# Autodesk Inventor assembly: Assembly1
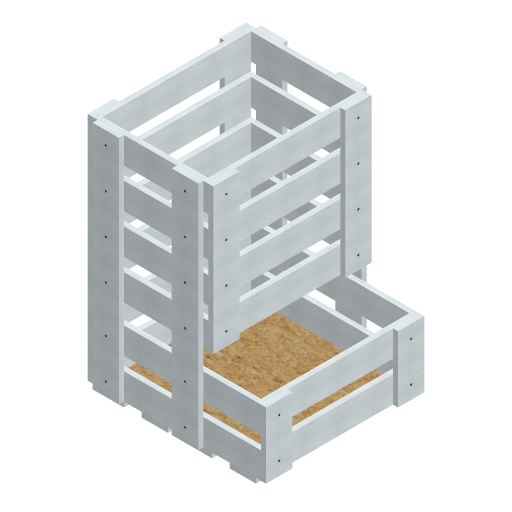
[picture p0: Inventor's stored thumbnail of the model, 512x512]
Saved by Autodesk Inventor 2024 (Build 280153000, 153)
## iProperties
Created: 2024-03-20
Part Number: Assembly1
Document SubType Name: Assembly
Designer: marco
Author: marco
## Documents named in this file (13)
- C:\Users\marco\OneDrive\Documents\FruitRack\Assembly1.iam
- C:\Users\marco\OneDrive\Documents\FruitRack\A.ipt
- C:\Users\marco\OneDrive\Documents\FruitRack\B.ipt
- C:\Users\marco\OneDrive\Documents\FruitRack\C.ipt
- C:\Users\marco\OneDrive\Documents\FruitRack\D.ipt
- C:\Users\marco\OneDrive\Documents\FruitRack\E.ipt
- C:\Users\marco\OneDrive\Documents\FruitRack\Screw.ipt
- C:\Users\marco\OneDrive\Documents\FruitRack\F.ipt
- C:\Users\marco\OneDrive\Documents\FruitRack\G.ipt
- C:\Users\marco\OneDrive\Documents\FruitRack\H.ipt
- C:\Users\marco\OneDrive\Documents\FruitRack\I.ipt
- C:\Users\marco\OneDrive\Documents\FruitRack\J.ipt
- C:\Users\marco\OneDrive\Documents\FruitRack\K.ipt
## Components (119 placed, 12 different names)
1. A:1 — Rigid:1, Rigid:2, Rigid:49, Rigid:68
2. A:2 — Rigid:3, Rigid:4, Rigid:50, Rigid:69
3. A:3 — Rigid:5, Rigid:6, Rigid:51, Rigid:70
4. A:4 — Rigid:7, Rigid:8, Rigid:52, Rigid:71
5. A:5 — Rigid:13, Rigid:14, Rigid:55, Rigid:62
6. A:6 — Rigid:15, Rigid:16, Rigid:56, Rigid:63
7. A:7 — Rigid:17, Rigid:18, Rigid:57, Rigid:64
8. A:8 — Rigid:19, Rigid:20, Rigid:58, Rigid:65
9. B:1 — Rigid:21, Rigid:22, Rigid:59, Rigid:66
10. B:2 — Rigid:9, Rigid:10, Rigid:53, Rigid:72
11. C:1 — Rigid:11, Rigid:12, Rigid:54, Rigid:73, Rigid:129, Rigid:130, Rigid:131, Rigid:132, Rigid:133
12. D:1 — Rigid:23, Rigid:24, Rigid:60, Rigid:67, Rigid:134, Rigid:135, Rigid:136, Rigid:137
13. E:1 — Rigid:25, Rigid:26, Rigid:27, Rigid:28, Rigid:29, Rigid:30
14. E:2 — Rigid:31, Rigid:32, Rigid:33, Rigid:34, Rigid:35, Rigid:36
15. E:3 — Rigid:43, Rigid:44, Rigid:45, Rigid:46, Rigid:47, Rigid:48
16. E:4 — Rigid:37, Rigid:38, Rigid:39, Rigid:40, Rigid:41, Rigid:42
17. Screw:1 — Rigid:1, Rigid:25
18. Screw:2 — Rigid:2, Rigid:31
19. Screw:3 — Rigid:3, Rigid:26
20. Screw:4 — Rigid:4, Rigid:32
21. Screw:5 — Rigid:5, Rigid:27
22. Screw:6 — Rigid:6, Rigid:33
23. Screw:7 — Rigid:7, Rigid:28
24. Screw:8 — Rigid:8, Rigid:34
25. Screw:9 — Rigid:9, Rigid:29
26. Screw:10 — Rigid:10, Rigid:35
27. Screw:11 — Rigid:11, Rigid:30
28. Screw:12 — Rigid:12, Rigid:36
29. Screw:13 — Rigid:13, Rigid:43
30. Screw:14 — Rigid:14, Rigid:37
31. Screw:15 — Rigid:15, Rigid:44
32. Screw:16 — Rigid:16, Rigid:38
33. Screw:17 — Rigid:17, Rigid:45
34. Screw:18 — Rigid:18, Rigid:39
35. Screw:19 — Rigid:19, Rigid:46
36. Screw:20 — Rigid:20, Rigid:40
37. Screw:21 — Rigid:21, Rigid:47
38. Screw:22 — Rigid:22, Rigid:41
39. Screw:23 — Rigid:23, Rigid:48
40. Screw:24 — Rigid:24, Rigid:42
41. F:1 — Rigid:74, Rigid:78, Rigid:87, Rigid:100
42. F:2 — Rotational:1, Rigid:79, Rigid:88, Rigid:94
43. F:3 — Rotational:2, Rigid:80, Rigid:89, Rigid:95
44. F:4 — Rigid:75, Rigid:90, Rigid:96
45. F:5 — Rigid:76, Rigid:91, Rigid:97
46. F:6 — Rigid:77, Rigid:98, Rigid:92
47. F:7 — Rotational:4, Rigid:110, Rigid:116
48. F:8 — Rigid:104, Rigid:111, Rigid:117
49. F:9 — Rigid:109, Rigid:112, Rigid:118
50. F:10 — Rigid:106, Rigid:113, Rigid:122
51. F:11 — Rigid:107, Rigid:114, Rigid:120
52. F:12 — Rigid:108, Rigid:115, Rigid:121
53. G:1 — Rigid:101
54. G:2 — Rigid:102
55. H:1 — Rotational:3
56. H:2 — Rigid:103
57. I:1 — Rigid:124, Rigid:125, Rigid:126, Rigid:127, Rigid:128
58. I:2 — Rigid:123
59. Screw:25 — Rigid:49, Rigid:74
60. Screw:26 — Rigid:50, Rotational:1
61. Screw:27 — Rigid:51, Rotational:2
62. Screw:28 — Rigid:52, Rigid:75
63. Screw:29 — Rigid:53, Rigid:76
64. Screw:30 — Rigid:54, Rigid:77
65. Screw:31 — Rigid:55, Rigid:78
66. Screw:32 — Rigid:56, Rigid:79
67. Screw:33 — Rigid:57, Rigid:80
68. Screw:34 — Rigid:58
69. Screw:35 — Rigid:59
70. Screw:36 — Rigid:60
71. Screw:37 — Rigid:68, Rotational:4
72. Screw:38 — Rigid:69, Rigid:104
73. Screw:39 — Rigid:70, Rigid:109
74. Screw:40 — Rigid:71, Rigid:106
75. Screw:41 — Rigid:72, Rigid:107
76. Screw:42 — Rigid:73, Rigid:108
77. Screw:43 — Rigid:63
78. Screw:44 — Rigid:62
79. Screw:45 — Rigid:64
80. Screw:46 — Rigid:65
81. Screw:47 — Rigid:66
82. Screw:48 — Rigid:67
83. Screw:49 — Rigid:87, Rigid:101
84. Screw:50 — Rigid:88
85. Screw:51 — Rigid:89
86. Screw:52 — Rigid:90
87. Screw:53 — Rigid:91, Rotational:3
88. Screw:54 — Rigid:92
89. Screw:55 — Rigid:100, Rigid:102
90. Screw:56 — Rigid:94
91. Screw:57 — Rigid:95
92. Screw:58 — Rigid:96
93. Screw:59 — Rigid:97, Rigid:103
94. Screw:60 — Rigid:98
95. Screw:61 — Rigid:110, Rigid:123
96. Screw:62 — Rigid:111
97. Screw:63 — Rigid:112
98. Screw:64 — Rigid:113
99. Screw:65 — Rigid:114
100. Screw:66 — Rigid:115
101. Screw:67 — Rigid:118, Rigid:127
102. Screw:68 — Rigid:116, Rigid:125
103. Screw:69 — Rigid:117, Rigid:126
104. Screw:70 — Rigid:122
105. Screw:71 — Rigid:120, Rigid:128
106. Screw:72 — Rigid:121, Rigid:124
107. J:1 — Rigid:138
108. J:2 — Rigid:139
109. J:3 — Rigid:140
110. J:4 — Rigid:141
111. K:1 — Rigid:129
112. Screw:73 — Rigid:130, Rigid:138
113. Screw:74 — Rigid:134
114. Screw:75 — Rigid:131, Rigid:139
115. Screw:76 — Rigid:135
116. Screw:77 — Rigid:132, Rigid:140
117. Screw:78 — Rigid:136
118. Screw:79 — Rigid:133, Rigid:141
119. Screw:80 — Rigid:137
## Relationships (134: WeldJoint 130, RevoluteJoint 4)
- Rigid:1 [WeldJoint] (11 mm): A:1 ↔ Screw:1
- Rigid:2 [WeldJoint] (11 mm): A:1 ↔ Screw:2
- Rigid:3 [WeldJoint] (11 mm): A:2 ↔ Screw:3
- Rigid:4 [WeldJoint] (11 mm): A:2 ↔ Screw:4
- Rigid:5 [WeldJoint] (11 mm): A:3 ↔ Screw:5
- Rigid:6 [WeldJoint] (11 mm): A:3 ↔ Screw:6
- Rigid:7 [WeldJoint] (11 mm): A:4 ↔ Screw:7
- Rigid:8 [WeldJoint] (11 mm): A:4 ↔ Screw:8
- Rigid:9 [WeldJoint] (11 mm): B:2 ↔ Screw:9
- Rigid:10 [WeldJoint] (11 mm): B:2 ↔ Screw:10
- Rigid:11 [WeldJoint] (11 mm): C:1 ↔ Screw:11
- Rigid:12 [WeldJoint] (11 mm): C:1 ↔ Screw:12
- Rigid:13 [WeldJoint] (11 mm): A:5 ↔ Screw:13
- Rigid:14 [WeldJoint] (11 mm): A:5 ↔ Screw:14
- Rigid:15 [WeldJoint] (11 mm): A:6 ↔ Screw:15
- Rigid:16 [WeldJoint] (11 mm): A:6 ↔ Screw:16
- Rigid:17 [WeldJoint] (11 mm): A:7 ↔ Screw:17
- Rigid:18 [WeldJoint] (11 mm): A:7 ↔ Screw:18
- Rigid:19 [WeldJoint] (11 mm): A:8 ↔ Screw:19
- Rigid:20 [WeldJoint] (11 mm): A:8 ↔ Screw:20
- Rigid:21 [WeldJoint] (11 mm): B:1 ↔ Screw:21
- Rigid:22 [WeldJoint] (11 mm): B:1 ↔ Screw:22
- Rigid:23 [WeldJoint] (11 mm): D:1 ↔ Screw:23
- Rigid:24 [WeldJoint] (11 mm): D:1 ↔ Screw:24
- Rigid:25 [WeldJoint]: E:1 ↔ Screw:1
- Rigid:26 [WeldJoint]: E:1 ↔ Screw:3
- Rigid:27 [WeldJoint]: E:1 ↔ Screw:5
- Rigid:28 [WeldJoint]: E:1 ↔ Screw:7
- Rigid:29 [WeldJoint]: E:1 ↔ Screw:9
- Rigid:30 [WeldJoint]: E:1 ↔ Screw:11
- Rigid:31 [WeldJoint]: E:2 ↔ Screw:2
- Rigid:32 [WeldJoint]: E:2 ↔ Screw:4
- Rigid:33 [WeldJoint]: E:2 ↔ Screw:6
- Rigid:34 [WeldJoint]: E:2 ↔ Screw:8
- Rigid:35 [WeldJoint]: E:2 ↔ Screw:10
- Rigid:36 [WeldJoint]: E:2 ↔ Screw:12
- Rigid:37 [WeldJoint]: E:4 ↔ Screw:14
- Rigid:38 [WeldJoint]: E:4 ↔ Screw:16
- Rigid:39 [WeldJoint]: E:4 ↔ Screw:18
- Rigid:40 [WeldJoint]: E:4 ↔ Screw:20
- Rigid:41 [WeldJoint]: E:4 ↔ Screw:22
- Rigid:42 [WeldJoint]: E:4 ↔ Screw:24
- Rigid:43 [WeldJoint]: E:3 ↔ Screw:13
- Rigid:44 [WeldJoint]: E:3 ↔ Screw:15
- Rigid:45 [WeldJoint]: E:3 ↔ Screw:17
- Rigid:46 [WeldJoint]: E:3 ↔ Screw:19
- Rigid:47 [WeldJoint]: E:3 ↔ Screw:21
- Rigid:48 [WeldJoint]: E:3 ↔ Screw:23
- Rigid:49 [WeldJoint]: A:1 ↔ Screw:25
- Rigid:50 [WeldJoint]: A:2 ↔ Screw:26
- Rigid:51 [WeldJoint]: A:3 ↔ Screw:27
- Rigid:52 [WeldJoint]: A:4 ↔ Screw:28
- Rigid:53 [WeldJoint]: B:2 ↔ Screw:29
- Rigid:54 [WeldJoint]: C:1 ↔ Screw:30
- Rigid:55 [WeldJoint]: A:5 ↔ Screw:31
- Rigid:56 [WeldJoint]: A:6 ↔ Screw:32
- Rigid:58 [WeldJoint]: A:8 ↔ Screw:34
- Rigid:59 [WeldJoint]: B:1 ↔ Screw:35
- Rigid:60 [WeldJoint]: D:1 ↔ Screw:36
- Rigid:57 [WeldJoint]: A:7 ↔ Screw:33
- Rigid:62 [WeldJoint]: A:5 ↔ Screw:44
- Rigid:63 [WeldJoint]: A:6 ↔ Screw:43
- Rigid:64 [WeldJoint]: A:7 ↔ Screw:45
- Rigid:65 [WeldJoint]: A:8 ↔ Screw:46
- Rigid:66 [WeldJoint]: B:1 ↔ Screw:47
- Rigid:67 [WeldJoint]: D:1 ↔ Screw:48
- Rigid:68 [WeldJoint]: A:1 ↔ Screw:37
- Rigid:69 [WeldJoint]: A:2 ↔ Screw:38
- Rigid:70 [WeldJoint]: A:3 ↔ Screw:39
- Rigid:71 [WeldJoint]: A:4 ↔ Screw:40
- Rigid:72 [WeldJoint]: B:2 ↔ Screw:41
- Rigid:73 [WeldJoint]: C:1 ↔ Screw:42
- Rigid:74 [WeldJoint]: F:1 ↔ Screw:25
- Rotational:1 [RevoluteJoint]: F:2 ↔ Screw:26
- Rotational:2 [RevoluteJoint]: F:3 ↔ Screw:27
- Rigid:75 [WeldJoint]: F:4 ↔ Screw:28
- Rigid:76 [WeldJoint]: F:5 ↔ Screw:29
- Rigid:77 [WeldJoint]: F:6 ↔ Screw:30
- Rigid:78 [WeldJoint]: F:1 ↔ Screw:31
- Rigid:79 [WeldJoint]: F:2 ↔ Screw:32
- Rigid:80 [WeldJoint]: F:3 ↔ Screw:33
- Rigid:87 [WeldJoint]: F:1 ↔ Screw:49
- Rigid:88 [WeldJoint]: F:2 ↔ Screw:50
- Rigid:89 [WeldJoint]: F:3 ↔ Screw:51
- Rigid:90 [WeldJoint]: F:4 ↔ Screw:52
- Rigid:91 [WeldJoint]: F:5 ↔ Screw:53
- Rigid:94 [WeldJoint]: F:2 ↔ Screw:56
- Rigid:95 [WeldJoint]: F:3 ↔ Screw:57
- Rigid:96 [WeldJoint]: F:4 ↔ Screw:58
- Rigid:97 [WeldJoint]: F:5 ↔ Screw:59
- Rigid:98 [WeldJoint]: F:6 ↔ Screw:60
- Rigid:92 [WeldJoint]: F:6 ↔ Screw:54
- Rigid:100 [WeldJoint]: F:1 ↔ Screw:55
- Rigid:101 [WeldJoint]: G:1 ↔ Screw:49
- Rigid:102 [WeldJoint]: G:2 ↔ Screw:55
- Rigid:103 [WeldJoint]: H:2 ↔ Screw:59
- Rotational:3 [RevoluteJoint]: H:1 ↔ Screw:53
- Rotational:4 [RevoluteJoint]: F:7 ↔ Screw:37
- Rigid:104 [WeldJoint]: F:8 ↔ Screw:38
- Rigid:106 [WeldJoint]: F:10 ↔ Screw:40
- Rigid:107 [WeldJoint]: F:11 ↔ Screw:41
- Rigid:108 [WeldJoint]: F:12 ↔ Screw:42
- Rigid:109 [WeldJoint]: F:9 ↔ Screw:39
- Rigid:110 [WeldJoint]: F:7 ↔ Screw:61
- Rigid:111 [WeldJoint]: F:8 ↔ Screw:62
- Rigid:112 [WeldJoint]: F:9 ↔ Screw:63
- Rigid:113 [WeldJoint]: F:10 ↔ Screw:64
- Rigid:114 [WeldJoint]: F:11 ↔ Screw:65
- Rigid:115 [WeldJoint]: F:12 ↔ Screw:66
- Rigid:116 [WeldJoint]: F:7 ↔ Screw:68
- Rigid:117 [WeldJoint]: F:8 ↔ Screw:69
- Rigid:118 [WeldJoint]: F:9 ↔ Screw:67
- Rigid:120 [WeldJoint]: F:11 ↔ Screw:71
- Rigid:121 [WeldJoint]: F:12 ↔ Screw:72
- Rigid:122 [WeldJoint]: F:10 ↔ Screw:70
- Rigid:123 [WeldJoint]: I:2 ↔ Screw:61
- Rigid:124 [WeldJoint]: I:1 ↔ Screw:72
- Rigid:125 [WeldJoint]: I:1 ↔ Screw:68
- Rigid:126 [WeldJoint]: I:1 ↔ Screw:69
- Rigid:127 [WeldJoint]: I:1 ↔ Screw:67
- Rigid:128 [WeldJoint]: I:1 ↔ Screw:71
- Rigid:129 [WeldJoint]: C:1 ↔ K:1
- Rigid:130 [WeldJoint]: C:1 ↔ Screw:73
- Rigid:131 [WeldJoint]: C:1 ↔ Screw:75
- Rigid:132 [WeldJoint]: C:1 ↔ Screw:77
- Rigid:133 [WeldJoint]: C:1 ↔ Screw:79
- Rigid:134 [WeldJoint]: D:1 ↔ Screw:74
- Rigid:135 [WeldJoint]: D:1 ↔ Screw:76
- Rigid:136 [WeldJoint]: D:1 ↔ Screw:78
- Rigid:137 [WeldJoint]: D:1 ↔ Screw:80
- Rigid:138 [WeldJoint]: J:1 ↔ Screw:73
- Rigid:139 [WeldJoint]: J:2 ↔ Screw:75
- Rigid:140 [WeldJoint]: J:3 ↔ Screw:77
- Rigid:141 [WeldJoint]: J:4 ↔ Screw:79
